# Autodesk Inventor assembly: POM_T5_01
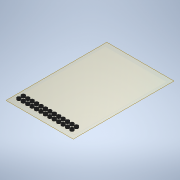
[picture p0: Inventor's stored thumbnail of the model, 180x180]
Saved by Autodesk Inventor 2020 (Build 240168000, 168)
## iProperties
Created: 2021-08-27
Part Number: POM_T5_01
Document SubType Name: Assembly
Designer: Masato
Author: Masato
## Documents named in this file (3)
- C:\Inventor\OpenPlatform_ver3_0\cam\POM_T5_01.iam
- C:\Inventor\OpenPlatform_ver3_0\cam\Disposable_Board.ipt
- C:\Inventor\OpenPlatform_ver3_0\Ready_Made\CC-0612-50B.ipt
## Components (27 placed, 2 different names)
1. Disposable_Board:1 — メイト:2, メイト:1, フラッシュ:1, フラッシュ:2, メイト:4, 正接:1, 正接:2, メイト:14, メイト:15, メイト:16, 正接:24, 正接:25, 正接:26, メイト:17, メイト:18, メイト:19, メイト:20, メイト:21, メイト:22, メイト:23, メイト:24, メイト:25, 正接:36, 正接:37, 正接:38, 正接:39, 正接:40, 正接:41, 正接:42, 正接:43, 正接:44
2. CC-0612-50B:1 — メイト:4, 正接:1, 正接:2, 正接:21
3. CC-0612-50B:11 — メイト:14, 正接:21, 正接:22, 正接:24
4. CC-0612-50B:12 — メイト:16, 正接:22, 正接:23, 正接:25
5. CC-0612-50B:13 — メイト:15, 正接:23, 正接:26, 正接:27
6. CC-0612-50B:16 — メイト:20, 正接:27, 正接:28, 正接:36
7. CC-0612-50B:21 — メイト:19, 正接:28, 正接:29, 正接:37
8. CC-0612-50B:15 — メイト:18, 正接:29, 正接:30, 正接:38
9. CC-0612-50B:17 — メイト:21, 正接:30, 正接:31, 正接:39
10. CC-0612-50B:22 — メイト:23, 正接:31, 正接:32, 正接:40
11. CC-0612-50B:19 — メイト:24, 正接:32, 正接:33, 正接:41
12. CC-0612-50B:18 — メイト:22, 正接:33, 正接:34, 正接:42
13. CC-0612-50B:20 — メイト:25, 正接:34, 正接:35, 正接:43
14. CC-0612-50B:14 — メイト:17, 正接:35, 正接:44
15. CC-0612-50B:23
16. CC-0612-50B:24
17. CC-0612-50B:25
18. CC-0612-50B:26
19. CC-0612-50B:27
20. CC-0612-50B:28
21. CC-0612-50B:29
22. CC-0612-50B:30
23. CC-0612-50B:31
24. CC-0612-50B:32
25. CC-0612-50B:33
26. CC-0612-50B:34
27. CC-0612-50B:35
## Component patterns: (2 elements, first: CC-0612-50B:1 + CC-0612-50B:11 + CC-0612-50B:12 + CC-0612-50B:13 + CC-0612-50B:16 + CC-0612-50B:21 + CC-0612-50B:15 + CC-0612-50B:17 + CC-0612-50B:22 + CC-0612-50B:19 + CC-0612-50B:18 + CC-0612-50B:20 + CC-0612-50B:14)
## Relationships (43: Tangent 26, Mate 15, Flush 2)
- メイト:2 [Mate]: Disposable_Board:1
- メイト:1 [Mate]: Disposable_Board:1
- フラッシュ:1 [Flush]: Disposable_Board:1
- フラッシュ:2 [Flush]: Disposable_Board:1
- メイト:4 [Mate]: Disposable_Board:1 ↔ CC-0612-50B:1
- 正接:1 [Tangent] (2.5 mm): Disposable_Board:1 ↔ CC-0612-50B:1
- 正接:2 [Tangent] (2.5 mm): Disposable_Board:1 ↔ CC-0612-50B:1
- メイト:14 [Mate]: Disposable_Board:1 ↔ CC-0612-50B:11
- メイト:15 [Mate]: Disposable_Board:1 ↔ CC-0612-50B:13
- メイト:16 [Mate]: Disposable_Board:1 ↔ CC-0612-50B:12
- 正接:21 [Tangent] (2.5 mm): CC-0612-50B:1 ↔ CC-0612-50B:11
- 正接:22 [Tangent] (2.5 mm): CC-0612-50B:11 ↔ CC-0612-50B:12
- 正接:23 [Tangent] (2.5 mm): CC-0612-50B:12 ↔ CC-0612-50B:13
- 正接:24 [Tangent] (2.5 mm): Disposable_Board:1 ↔ CC-0612-50B:11
- 正接:25 [Tangent] (2.5 mm): Disposable_Board:1 ↔ CC-0612-50B:12
- 正接:26 [Tangent] (2.5 mm): Disposable_Board:1 ↔ CC-0612-50B:13
- メイト:17 [Mate]: Disposable_Board:1 ↔ CC-0612-50B:14
- メイト:18 [Mate]: Disposable_Board:1 ↔ CC-0612-50B:15
- メイト:19 [Mate]: Disposable_Board:1 ↔ CC-0612-50B:21
- メイト:20 [Mate]: Disposable_Board:1 ↔ CC-0612-50B:16
- メイト:21 [Mate]: Disposable_Board:1 ↔ CC-0612-50B:17
- メイト:22 [Mate]: Disposable_Board:1 ↔ CC-0612-50B:18
- メイト:23 [Mate]: Disposable_Board:1 ↔ CC-0612-50B:22
- メイト:24 [Mate]: Disposable_Board:1 ↔ CC-0612-50B:19
- メイト:25 [Mate]: Disposable_Board:1 ↔ CC-0612-50B:20
- 正接:27 [Tangent] (2.5 mm): CC-0612-50B:13 ↔ CC-0612-50B:16
- 正接:28 [Tangent] (2.5 mm): CC-0612-50B:16 ↔ CC-0612-50B:21
- 正接:29 [Tangent] (2.5 mm): CC-0612-50B:21 ↔ CC-0612-50B:15
- 正接:30 [Tangent] (2.5 mm): CC-0612-50B:15 ↔ CC-0612-50B:17
- 正接:31 [Tangent] (2.5 mm): CC-0612-50B:17 ↔ CC-0612-50B:22
- 正接:32 [Tangent] (2.5 mm): CC-0612-50B:22 ↔ CC-0612-50B:19
- 正接:33 [Tangent] (2.5 mm): CC-0612-50B:19 ↔ CC-0612-50B:18
- 正接:34 [Tangent] (2.5 mm): CC-0612-50B:18 ↔ CC-0612-50B:20
- 正接:35 [Tangent] (2.5 mm): CC-0612-50B:20 ↔ CC-0612-50B:14
- 正接:36 [Tangent] (2.5 mm): Disposable_Board:1 ↔ CC-0612-50B:16
- 正接:37 [Tangent] (2.5 mm): Disposable_Board:1 ↔ CC-0612-50B:21
- 正接:38 [Tangent] (2.5 mm): Disposable_Board:1 ↔ CC-0612-50B:15
- 正接:39 [Tangent] (2.5 mm): Disposable_Board:1 ↔ CC-0612-50B:17
- 正接:40 [Tangent] (2.5 mm): Disposable_Board:1 ↔ CC-0612-50B:22
- 正接:41 [Tangent] (2.5 mm): Disposable_Board:1 ↔ CC-0612-50B:19
- 正接:42 [Tangent] (2.5 mm): Disposable_Board:1 ↔ CC-0612-50B:18
- 正接:43 [Tangent] (2.5 mm): Disposable_Board:1 ↔ CC-0612-50B:20
- 正接:44 [Tangent] (2.5 mm): Disposable_Board:1 ↔ CC-0612-50B:14
